# Autodesk Inventor assembly: bottom
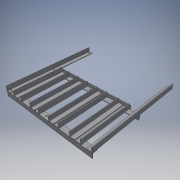
[picture p0: Inventor's stored thumbnail of the model, 180x180]
Saved by Autodesk Inventor 2017 (Build 210142000, 142)
## iProperties
Created: 2018-10-17
Part Number: bottom
Document SubType Name: Assembly
Designer: ddeboer
Author: ddeboer
## Documents named in this file (4)
- C:\Users\ddeboer\Desktop\snap_holder\bottom.iam
- C:\Users\ddeboer\Desktop\snap_holder\ladder.iam
- C:\Users\ddeboer\Desktop\snap_holder\channel.ipt
- C:\Users\ddeboer\Desktop\snap_holder\backstop.ipt
## Components (4 placed, 3 different names)
1. ladder:1 [sub-assembly] — Insert:1, Flush:1, Insert:2, Mate:1, Flush:2
2. channel:1 — Insert:1, Flush:1
3. channel:2 — Insert:2, Flush:2
4. backstop:1 — Mate:1
## Relationships (5: Insert 2, Flush 2, Mate 1)
- Insert:1: ladder:1 ↔ channel:1
- Flush:1: ladder:1 ↔ channel:1
- Insert:2: ladder:1 ↔ channel:2
- Mate:1: ladder:1 ↔ backstop:1
- Flush:2: ladder:1 ↔ channel:2
